# Autodesk Inventor assembly: ENSAMBLE_RECICLADOR
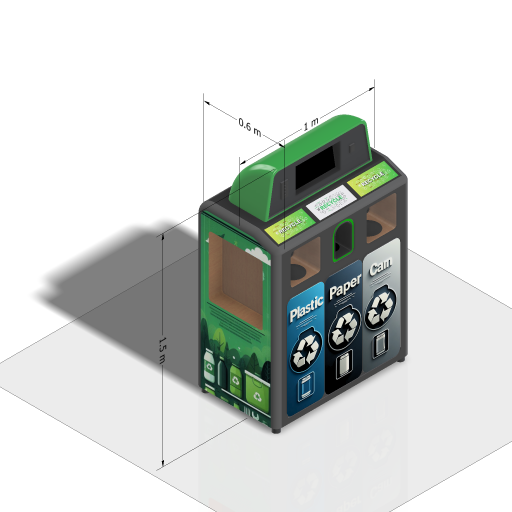
[picture p0: Inventor's stored thumbnail of the model, 512x512]
Saved by Autodesk Inventor 2024.1 (Build 281209000, 209)
## iProperties
Created: 2024-04-17
Part Number: ENSAMBLE_RECICLADOR
Material: Generic
Document SubType Name: Assembly
Designer: Niler
Author: Niler
## Documents named in this file (4)
- C:\Users\Niler\OneDrive\Escritorio\RECICLADOR\ENSAMBLE_RECICLADOR.iam
- C:\Users\Niler\OneDrive\Escritorio\RECICLADOR\CARCASA_V1.ipt
- C:\Users\Niler\OneDrive\Escritorio\RECICLADOR\VIDRIO.ipt
- C:\Users\Niler\OneDrive\Escritorio\RECICLADOR\VIDRIO2.ipt
## Components (4 placed, 3 different names)
1. CARCASA_V1:1 — Mate:1, Flush:1, Mate:2, Mate:3, Mate:4, Flush:2, Mate:5, Mate:6, Flush:3
2. VIDRIO:1 — Mate:3, Mate:4, Flush:2
3. VIDRIO2:1 — Mate:5, Mate:6, Flush:3
4. VIDRIO2:2 — Mate:1, Flush:1, Mate:2
## Relationships (9: Mate 6, Flush 3)
- Mate:1: CARCASA_V1:1 ↔ VIDRIO2:2
- Flush:1: CARCASA_V1:1 ↔ VIDRIO2:2
- Mate:2: CARCASA_V1:1 ↔ VIDRIO2:2
- Mate:3: CARCASA_V1:1 ↔ VIDRIO:1
- Mate:4: CARCASA_V1:1 ↔ VIDRIO:1
- Flush:2: CARCASA_V1:1 ↔ VIDRIO:1
- Mate:5: CARCASA_V1:1 ↔ VIDRIO2:1
- Mate:6: CARCASA_V1:1 ↔ VIDRIO2:1
- Flush:3: CARCASA_V1:1 ↔ VIDRIO2:1
